# Autodesk Inventor assembly: Редуктор в сборе
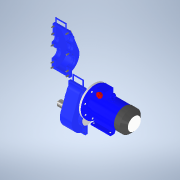
[picture p0: Inventor's stored thumbnail of the model, 180x180]
Saved by Autodesk Inventor 2021 (Build 250183000, 183)
## iProperties
Created: 2023-03-03
Part Number: Редуктор в сборе
Document SubType Name: Assembly
Designer: gdevc
Mass: 9249.32 g
Surface Area: 2771.27 cm^2
Volume: 1186.1 cm^3
Density: 7.79807 g/cm^3
Author: gdevc
## Documents named in this file (24)
- C:\Users\gdevc\OneDrive\Рабочий стол\Курсач\DetaliMashine\Новая папка\Редуктор в сборе.iam
- C:\Users\gdevc\OneDrive\Рабочий стол\Курсач\DetaliMashine\Новая папка\Вал_промежуточный.ipt
- C:\Users\gdevc\OneDrive\Рабочий стол\Курсач\DetaliMashine\Новая папка\Редуктор в сборе\Мастер проектирования\Цилиндрическое зубчатое зацепление1.iam
- C:\Users\gdevc\OneDrive\Рабочий стол\Курсач\DetaliMashine\Новая папка\Колесо быстроходное.ipt
- C:\Users\gdevc\OneDrive\Рабочий стол\Курсач\DetaliMashine\Новая папка\Редуктор в сборе\Мастер проектирования\Цилиндрическое зубчатое зацепление2.iam
- C:\Users\gdevc\OneDrive\Рабочий стол\Курсач\DetaliMashine\Новая папка\Вал_тихоходный.ipt
- C:\Users\gdevc\OneDrive\Рабочий стол\Курсач\DetaliMashine\Новая папка\Редуктор в сборе\Мастер проектирования\Цилиндрическое зубчатое зацепление3.iam
- C:\Users\gdevc\OneDrive\Рабочий стол\Курсач\DetaliMashine\Новая папка\Валл быстроходный.ipt
- C:\Users\gdevc\OneDrive\Рабочий стол\Курсач\DetaliMashine\Новая папка\Редуктор в сборе\Мастер проектирования\Цилиндрическое зубчатое зацепление4.iam
- C:\Users\gdevc\OneDrive\Рабочий стол\Курсач\DetaliMashine\Новая папка\Крышка тих_выход.ipt
- C:\Users\gdevc\OneDrive\Рабочий стол\Курсач\DetaliMashine\Новая папка\Крышка, тихая.ipt
- C:\Users\gdevc\OneDrive\Рабочий стол\Курсач\DetaliMashine\Новая папка\Крышка_пром.ipt
- C:\Users\gdevc\OneDrive\Рабочий стол\Курсач\DetaliMashine\Новая папка\Корпус.v.2.0.iam
- C:\Users\gdevc\OneDrive\Рабочий стол\Курсач\DetaliMashine\Новая папка\Манжет 1-30x47x7 ГОСТ 8752-79.ipt
- C:\Users\gdevc\OneDrive\Рабочий стол\Курсач\DetaliMashine\Новая папка\Крышка_быстроходного.ipt
- C:\Users\gdevc\OneDrive\Рабочий стол\Курсач\DetaliMashine\Новая папка\Подшипник 210 ГОСТ 8338-75.ipt
- C:\Users\gdevc\OneDrive\Рабочий стол\Курсач\DetaliMashine\Новая папка\Подшипник 205 ГОСТ 8338-75.ipt
- C:\Users\gdevc\OneDrive\Рабочий стол\Курсач\DetaliMashine\Новая папка\Манжет 2-50x65x8 ГОСТ 8752-79.ipt
- C:\Users\gdevc\OneDrive\Рабочий стол\Курсач\DetaliMashine\Новая папка\Болт M10×35 ГОСТ Р 50793-95.ipt
- C:\Users\gdevc\OneDrive\Рабочий стол\Курсач\DetaliMashine\Новая папка\Промежуточное колесо резина.ipt
- C:\Users\gdevc\OneDrive\Рабочий стол\Курсач\DetaliMashine\Новая папка\Редуктор в сборе\Мастер проектирования\Цилиндрическое зубчатое зацепление5.iam
- C:\Users\gdevc\OneDrive\Рабочий стол\Курсач\DetaliMashine\Новая папка\Резина конец.ipt
- C:\Users\gdevc\OneDrive\Рабочий стол\Курсач\DetaliMashine\Новая папка\Редуктор в сборе\Мастер проектирования\Цилиндрическое зубчатое зацепление6.iam
- C:\Users\gdevc\Downloads\Telegram Desktop\АИР100L IM2081 (2,4,6,8 пол)....ipt
## Components (34 placed, 18 different names)
1. Вал_промежуточный:1 — Совмещение:2, Совмещение:4, Совмещение:5, Совмещение:9, Заподлицо:2, Совмещение:14, Совмещение:15, Совмещение:16, Совмещение:17, Симметрия:1, Совмещение:25, Совмещение:27
2. Цилиндрическое зубчатое зацепление:1 [sub-assembly]
3. Колесо быстроходное:1 — Совмещение:4, Совмещение:5, Заподлицо:3, Заподлицо:4
4. Цилиндрическое зубчатое зацепление:2 [sub-assembly]
5. Вал_тихоходный:1 — Совмещение:9, Заподлицо:2, Совмещение:10, Совмещение:11, Совмещение:12, Совмещение:13, Совмещение:18, Совмещение:21, Совмещение:23, Совмещение:29, Совмещение:55
6. Цилиндрическое зубчатое зацепление:3 [sub-assembly]
7. Валл быстроходный:1 — Совмещение:2, Заподлицо:3, Совмещение:32, Угол:3, Совмещение:36, Совмещение:56
8. Цилиндрическое зубчатое зацепление:4 [sub-assembly]
9. Подшипник 205 ГОСТ 8338-75:1 — Совмещение:14, Совмещение:15, Симметрия:1, Совмещение:26
10. Подшипник 205 ГОСТ 8338-75:2 — Совмещение:16, Совмещение:17, Совмещение:28
11. Подшипник 210 ГОСТ 8338-75:1 — Совмещение:10, Совмещение:11
12. Подшипник 210 ГОСТ 8338-75:2 — Совмещение:12, Совмещение:13, Совмещение:30
13. Манжет 2-50x65x8 ГОСТ 8752-79:1 — Совмещение:18
14. Крышка тих_выход:1 — Совмещение:21, Совмещение:30
15. Крышка, тихая:1 — Совмещение:23, Совмещение:35
16. Крышка_пром:1 — Совмещение:25, Совмещение:26
17. Крышка_пром:2 — Совмещение:27, Совмещение:28, Совмещение:31
18. Корпус.v.2.0:1 [sub-assembly] — Совмещение:29, Угол:2, Совмещение:31, Совмещение:34, Совмещение:35, Совмещение:37, Совмещение:38, Совмещение:39, Совмещение:40, Совмещение:41, Совмещение:42, Совмещение:43, Совмещение:44, Совмещение:45, Совмещение:46, Совмещение:47, Совмещение:48, Совмещение:49, Совмещение:50, Совмещение:51, Совмещение:52, Совмещение:53, Совмещение:54
19. Манжет 1-30x47x7 ГОСТ 8752-79:1 — Совмещение:32, Совмещение:33
20. Крышка_быстроходного:1 — Совмещение:33, Совмещение:34, Совмещение:57
21. Болт M10×35 ГОСТ Р 50793-95:1 — Совмещение:37, Совмещение:46
22. Болт M10×35 ГОСТ Р 50793-95:2 — Совмещение:38, Совмещение:47
23. Болт M10×35 ГОСТ Р 50793-95:3 — Совмещение:39, Совмещение:49
24. Болт M10×35 ГОСТ Р 50793-95:4 — Совмещение:40, Совмещение:48
25. Болт M10×35 ГОСТ Р 50793-95:5 — Совмещение:41, Совмещение:51
26. Болт M10×35 ГОСТ Р 50793-95:6 — Совмещение:42, Совмещение:53
27. Болт M10×35 ГОСТ Р 50793-95:7 — Совмещение:43, Совмещение:50
28. Болт M10×35 ГОСТ Р 50793-95:8 — Совмещение:44, Совмещение:52
29. Болт M10×35 ГОСТ Р 50793-95:9 — Совмещение:45, Совмещение:54
30. Промежуточное колесо резина:1 — Совмещение:55, Заподлицо:4
31. Цилиндрическое зубчатое зацепление:5 [sub-assembly]
32. Резина конец:1
33. Цилиндрическое зубчатое зацепление:6 [sub-assembly]
34. АИР100L IM2081 (2,4,6,8 пол)...:1 — Совмещение:56, Совмещение:57
## Relationships (54: Mate 48, Flush 3, Angle 2, Symmetry 1)
- Совмещение:2 [Mate] (63 mm): Вал_промежуточный:1 ↔ Валл быстроходный:1
- Совмещение:4 [Mate]: Вал_промежуточный:1 ↔ Колесо быстроходное:1
- Совмещение:5 [Mate]: Вал_промежуточный:1 ↔ Колесо быстроходное:1
- Совмещение:9 [Mate] (-100 mm): Вал_промежуточный:1 ↔ Вал_тихоходный:1
- Заподлицо:2 [Flush] (1.5 mm): Вал_промежуточный:1 ↔ Вал_тихоходный:1
- Совмещение:10 [Mate]: Вал_тихоходный:1 ↔ Подшипник 210 ГОСТ 8338-75:1
- Совмещение:11 [Mate]: Вал_тихоходный:1 ↔ Подшипник 210 ГОСТ 8338-75:1
- Совмещение:12 [Mate]: Вал_тихоходный:1 ↔ Подшипник 210 ГОСТ 8338-75:2
- Совмещение:13 [Mate]: Вал_тихоходный:1 ↔ Подшипник 210 ГОСТ 8338-75:2
- Совмещение:14 [Mate]: Вал_промежуточный:1 ↔ Подшипник 205 ГОСТ 8338-75:1
- Совмещение:15 [Mate]: Вал_промежуточный:1 ↔ Подшипник 205 ГОСТ 8338-75:1
- Совмещение:16 [Mate]: Вал_промежуточный:1 ↔ Подшипник 205 ГОСТ 8338-75:2
- Совмещение:17 [Mate]: Вал_промежуточный:1 ↔ Подшипник 205 ГОСТ 8338-75:2
- Совмещение:18 [Mate]: Вал_тихоходный:1 ↔ Манжет 2-50x65x8 ГОСТ 8752-79:1
- Симметрия:1 [Symmetry]: Вал_промежуточный:1 ↔ Подшипник 205 ГОСТ 8338-75:1
- Совмещение:21 [Mate]: Вал_тихоходный:1 ↔ Крышка тих_выход:1
- Совмещение:23 [Mate]: Вал_тихоходный:1 ↔ Крышка, тихая:1
- Совмещение:25 [Mate]: Вал_промежуточный:1 ↔ Крышка_пром:1
- Совмещение:26 [Mate]: Подшипник 205 ГОСТ 8338-75:1 ↔ Крышка_пром:1
- Совмещение:27 [Mate]: Вал_промежуточный:1 ↔ Крышка_пром:2
- Совмещение:28 [Mate]: Подшипник 205 ГОСТ 8338-75:2 ↔ Крышка_пром:2
- Совмещение:29 [Mate]: Вал_тихоходный:1 ↔ Корпус.v.2.0:1
- Угол:2 [Angle] (90 deg): Корпус.v.2.0:1
- Совмещение:30 [Mate]: Подшипник 210 ГОСТ 8338-75:2 ↔ Крышка тих_выход:1
- Совмещение:31 [Mate]: Крышка_пром:2 ↔ Корпус.v.2.0:1
- Заподлицо:3 [Flush] (-1 mm): Колесо быстроходное:1 ↔ Валл быстроходный:1
- Совмещение:32 [Mate]: Валл быстроходный:1 ↔ Манжет 1-30x47x7 ГОСТ 8752-79:1
- Совмещение:33 [Mate]: Манжет 1-30x47x7 ГОСТ 8752-79:1 ↔ Крышка_быстроходного:1
- Совмещение:34 [Mate]: Корпус.v.2.0:1 ↔ Крышка_быстроходного:1
- Совмещение:35 [Mate]: Крышка, тихая:1 ↔ Корпус.v.2.0:1
- Угол:3 [Angle] (90 deg): Валл быстроходный:1
- Совмещение:36 [Mate]: Валл быстроходный:1
- Совмещение:37 [Mate]: Корпус.v.2.0:1 ↔ Болт M10×35 ГОСТ Р 50793-95:1
- Совмещение:38 [Mate]: Корпус.v.2.0:1 ↔ Болт M10×35 ГОСТ Р 50793-95:2
- Совмещение:39 [Mate]: Корпус.v.2.0:1 ↔ Болт M10×35 ГОСТ Р 50793-95:3
- Совмещение:40 [Mate]: Корпус.v.2.0:1 ↔ Болт M10×35 ГОСТ Р 50793-95:4
- Совмещение:41 [Mate]: Корпус.v.2.0:1 ↔ Болт M10×35 ГОСТ Р 50793-95:5
- Совмещение:42 [Mate]: Корпус.v.2.0:1 ↔ Болт M10×35 ГОСТ Р 50793-95:6
- Совмещение:43 [Mate]: Корпус.v.2.0:1 ↔ Болт M10×35 ГОСТ Р 50793-95:7
- Совмещение:44 [Mate]: Корпус.v.2.0:1 ↔ Болт M10×35 ГОСТ Р 50793-95:8
- Совмещение:45 [Mate]: Корпус.v.2.0:1 ↔ Болт M10×35 ГОСТ Р 50793-95:9
- Совмещение:46 [Mate]: Корпус.v.2.0:1 ↔ Болт M10×35 ГОСТ Р 50793-95:1
- Совмещение:47 [Mate]: Корпус.v.2.0:1 ↔ Болт M10×35 ГОСТ Р 50793-95:2
- Совмещение:48 [Mate]: Корпус.v.2.0:1 ↔ Болт M10×35 ГОСТ Р 50793-95:4
- Совмещение:49 [Mate]: Корпус.v.2.0:1 ↔ Болт M10×35 ГОСТ Р 50793-95:3
- Совмещение:50 [Mate]: Корпус.v.2.0:1 ↔ Болт M10×35 ГОСТ Р 50793-95:7
- Совмещение:51 [Mate]: Корпус.v.2.0:1 ↔ Болт M10×35 ГОСТ Р 50793-95:5
- Совмещение:52 [Mate]: Корпус.v.2.0:1 ↔ Болт M10×35 ГОСТ Р 50793-95:8
- Совмещение:53 [Mate]: Корпус.v.2.0:1 ↔ Болт M10×35 ГОСТ Р 50793-95:6
- Совмещение:54 [Mate]: Корпус.v.2.0:1 ↔ Болт M10×35 ГОСТ Р 50793-95:9
- Совмещение:55 [Mate]: Вал_тихоходный:1 ↔ Промежуточное колесо резина:1
- Заподлицо:4 [Flush] (-1 mm): Колесо быстроходное:1 ↔ Промежуточное колесо резина:1
- Совмещение:56 [Mate]: Валл быстроходный:1 ↔ АИР100L IM2081 (2,4,6,8 пол)...:1
- Совмещение:57 [Mate]: Крышка_быстроходного:1 ↔ АИР100L IM2081 (2,4,6,8 пол)...:1
